# Autodesk Inventor assembly: weldedAssembly
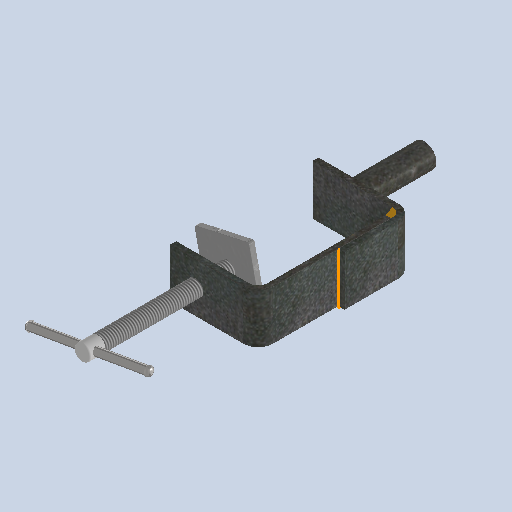
[picture p0: Inventor's stored thumbnail of the model, 512x512]
Saved by Autodesk Inventor 2024.2 (Build 282272000, 272)
## iProperties
Created: 2024-05-25
Part Number: weldedAssembly
Document SubType Name: Weldment
Designer: user
Weld Material: Stainless Steel AISI 440C, Welded
Author: user
## Documents named in this file (7)
- D:\Users\user\Documents\CAD\2024\Maize sheller Version2\weldedClampAssembly.iam
- D:\Users\user\Documents\CAD\2024\Maize sheller Version2\clampBaseBottom.ipt
- D:\Users\user\Documents\CAD\2024\Maize sheller Version2\clampBaseTopSide.ipt
- D:\Users\user\Documents\CAD\2024\Maize sheller Version2\connecting shaft.ipt
- D:\Users\user\Documents\CAD\2024\Maize sheller Version2\clampScrew.ipt
- D:\Users\user\Documents\CAD\2024\Maize sheller Version2\clampPlate.ipt
- D:\Users\user\Documents\CAD\2024\Maize sheller Version2\clampScrewHandle.ipt
## Components (6 placed, 6 different names)
1. clampBaseBottom:1 — Mate:1, Flush:1, Mate:4, Mate:5, Tangent:1, Mate:8, Flush:2
2. clampBaseTopSide:1 — Mate:2, Mate:5, Tangent:1, Mate:6, Mate:7
3. connecting shaft:1 — Mate:3, Mate:6, Mate:7
4. clampScrew:1 — Mate:8, Flush:2, Mate:9, Flush:3, Mate:10, Mate:11
5. clampPlate:1 — Mate:9, Flush:3
6. clampScrewHandle:1 — Mate:10, Mate:11
## Relationships (15: Mate 11, Flush 3, Tangent 1)
- Mate:1: clampBaseBottom:1
- Mate:2: clampBaseTopSide:1
- Mate:3: connecting shaft:1
- Flush:1: clampBaseBottom:1
- Mate:4: clampBaseBottom:1
- Mate:5: clampBaseBottom:1 ↔ clampBaseTopSide:1
- Tangent:1: clampBaseBottom:1 ↔ clampBaseTopSide:1
- Mate:6: clampBaseTopSide:1 ↔ connecting shaft:1
- Mate:7: clampBaseTopSide:1 ↔ connecting shaft:1
- Mate:8: clampBaseBottom:1 ↔ clampScrew:1
- Flush:2 (-50 mm): clampBaseBottom:1 ↔ clampScrew:1
- Mate:9: clampScrew:1 ↔ clampPlate:1
- Flush:3: clampScrew:1 ↔ clampPlate:1
- Mate:10: clampScrew:1 ↔ clampScrewHandle:1
- Mate:11: clampScrew:1 ↔ clampScrewHandle:1
